# Autodesk Inventor assembly: Chain Drive
Saved by Autodesk Inventor 2016 SP1 (Build 200210100, 210)
## iProperties
Created: 2016-02-02
Part Number: Chain Drive
Document SubType Name: Assembly
Designer: steele
Mass: 308.319 g
Surface Area: 1242.62 cm^2
Volume: 196.511 cm^3
Density: 1.56896 g/cm^3
ClientObjectVersion: 1
Author: steele
## Documents named in this file (4)
- C:\snobotics\CAD-Development\robSteele\SnoBotics2016\2016-01-31-Lift\TelescopingArm\Design Accelerator\Chain Drive1.iam
- C:\snobotics\CAD-Development\robSteele\SnoBotics2016\2016-01-31-Lift\TelescopingArm\Design Accelerator\Roller Chain1.ipt
- C:\snobotics\CAD-Development\robSteele\SnoBotics2016\2016-01-31-Lift\TelescopingArm\Design Accelerator\Roller Chain Sprocket11.ipt
- C:\snobotics\CAD-Development\robSteele\SnoBotics2016\2016-01-31-Lift\TelescopingArm\Design Accelerator\Roller Chain Sprocket21.ipt
## Components (3 placed, 3 different names)
1. Roller Chain:1 — Flush:1, Mate:1, Mate:2, Flush:2, Mate:3, Mate:4
2. Roller Chain Sprocket1:1 — Flush:1, Mate:1, Mate:2, Rotation:1
3. Roller Chain Sprocket2:1 — Flush:2, Mate:3, Rotation:1, Mate:4
## Relationships (7: Mate 4, Flush 2, RelateRotation 1)
- Flush:1: Roller Chain:1 ↔ Roller Chain Sprocket1:1
- Mate:1: Roller Chain:1 ↔ Roller Chain Sprocket1:1
- Mate:2: Roller Chain:1 ↔ Roller Chain Sprocket1:1
- Flush:2: Roller Chain:1 ↔ Roller Chain Sprocket2:1
- Mate:3: Roller Chain:1 ↔ Roller Chain Sprocket2:1
- Rotation:1 [RelateRotation] (1 ul): Roller Chain Sprocket1:1 ↔ Roller Chain Sprocket2:1
- Mate:4: Roller Chain:1 ↔ Roller Chain Sprocket2:1
